# Autodesk Inventor assembly: TEST SCREW ARM
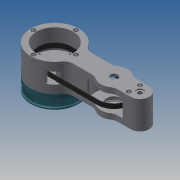
[picture p0: Inventor's stored thumbnail of the model, 180x180]
Saved by Autodesk Inventor 2013 (Build 170138000, 138)
## iProperties
Created: 2017-04-04
Part Number: TEST SCREW ARM
Document SubType Name: Assembly
Designer: employee
Author: employee
## Documents named in this file (10)
- C:\Users\employee\Desktop\SCARA\TEST SCREW ARM.iam
- C:\Users\employee\Desktop\SCARA\SCREW BOTTOM ARM.ipt
- C:\Users\employee\Desktop\SCARA\SCREW TOP ARM.ipt
- C:\Users\employee\Desktop\SCARA\lm6luu.ipt
- C:\Users\employee\Desktop\SCARA\distal drive pulley.ipt
- C:\Users\employee\Desktop\SCARA\M3x35.ipt
- C:\Users\employee\Desktop\SCARA\M3x30.ipt
- C:\Users\employee\Desktop\SCARA\608 bearing.ipt
- C:\Users\employee\Desktop\SCARA\washer.ipt
- C:\Users\employee\Desktop\SCARA\Z belt.ipt
## Components (18 placed, 9 different names)
1. SCREW BOTTOM ARM:1 — Mate:1, Insert:11, Mate:6
2. SCREW TOP ARM:1 — Mate:1, Insert:3, Insert:4, Insert:5, Insert:6, Insert:7, Insert:8, Insert:9, Insert:10, Mate:2, Insert:11, Mate:3, Insert:20
3. lm6luu:1 — Insert:3
4. distal drive pulley:1 — Insert:10, Mate:2, Mate:3, Insert:12, Insert:13, Insert:14, Insert:15, Insert:19
5. M3x35:1 — Insert:7
6. M3x35:2 — Insert:6
7. M3x35:3 — Insert:5
8. M3x35:4 — Insert:4
9. M3x35:5 — Insert:9
10. M3x35:6 — Insert:8
11. M3x30:1 — Insert:12
12. M3x30:2 — Insert:14
13. M3x30:3 — Insert:15
14. M3x30:4 — Insert:13
15. 608 bearing:1 — Insert:19
16. 608 bearing:2 — Insert:20, Insert:21
17. washer:1 — Insert:21
18. Z belt:1 — Mate:6
## Relationships (20: Insert 16, Mate 4)
- Mate:1: SCREW BOTTOM ARM:1 ↔ SCREW TOP ARM:1
- Insert:3: SCREW TOP ARM:1 ↔ lm6luu:1
- Insert:4: SCREW TOP ARM:1 ↔ M3x35:4
- Insert:5: SCREW TOP ARM:1 ↔ M3x35:3
- Insert:6: SCREW TOP ARM:1 ↔ M3x35:2
- Insert:7: SCREW TOP ARM:1 ↔ M3x35:1
- Insert:8: SCREW TOP ARM:1 ↔ M3x35:6
- Insert:9: SCREW TOP ARM:1 ↔ M3x35:5
- Insert:10: SCREW TOP ARM:1 ↔ distal drive pulley:1
- Mate:2: SCREW TOP ARM:1 ↔ distal drive pulley:1
- Insert:11: SCREW BOTTOM ARM:1 ↔ SCREW TOP ARM:1
- Mate:3: SCREW TOP ARM:1 ↔ distal drive pulley:1
- Insert:12: distal drive pulley:1 ↔ M3x30:1
- Insert:13: distal drive pulley:1 ↔ M3x30:4
- Insert:14: distal drive pulley:1 ↔ M3x30:2
- Insert:15: distal drive pulley:1 ↔ M3x30:3
- Insert:19: distal drive pulley:1 ↔ 608 bearing:1
- Insert:20: SCREW TOP ARM:1 ↔ 608 bearing:2
- Insert:21: 608 bearing:2 ↔ washer:1
- Mate:6: SCREW BOTTOM ARM:1 ↔ Z belt:1
